# Autodesk Inventor assembly: motor_block
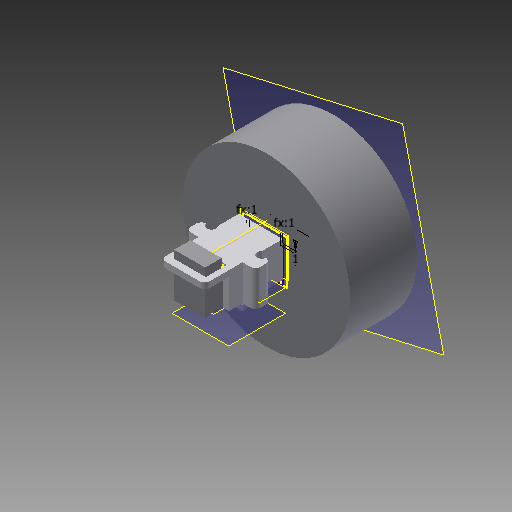
[picture p0: Inventor's stored thumbnail of the model, 512x512]
Saved by Autodesk Inventor 2018 (Build 220112000, 112)
## iProperties
Created: 2017-09-28
Part Number: motor_block
Document SubType Name: Assembly
Designer: fabre
Author: fabre
## Documents named in this file (4)
- C:\Users\rfabre\Desktop\cubi\mechanics\pendulum\motor_block.iam
- C:\Users\rfabre\Desktop\cubi\mechanics\pendulum\motor.ipt
- C:\Users\rfabre\Desktop\cubi\mechanics\pendulum\motorbox_unique.ipt
- C:\Users\rfabre\Desktop\cubi\mechanics\pendulum\wheel.ipt
## Components (3 placed, 3 different names)
1. motor:1 — Mate:1, Mate:2, Mate:3, Mate:4, Mate:5, Mate:6
2. motorbox_unique:1 — Mate:1, Mate:2, Mate:3, Mate:4
3. wheel:1 — Mate:5, Mate:6
## Relationships (6: Mate 6)
- Mate:1: motor:1 ↔ motorbox_unique:1
- Mate:2: motor:1 ↔ motorbox_unique:1
- Mate:3: motor:1 ↔ motorbox_unique:1
- Mate:4: motor:1 ↔ motorbox_unique:1
- Mate:5: motor:1 ↔ wheel:1
- Mate:6 (1 mm): motor:1 ↔ wheel:1
